# Autodesk Inventor assembly: Motor assembly V2
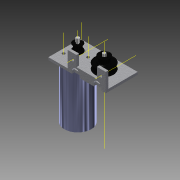
[picture p0: Inventor's stored thumbnail of the model, 180x180]
Saved by Autodesk Inventor 2013 (Build 170138000, 138)
## iProperties
Created: 2013-01-03
Part Number: Motor assembly V2
Document SubType Name: Assembly
Designer: Nico
Author: Nico
## Documents named in this file (5)
- D:\Documents\Inventor\Coil winder\IAM files\Motor assembly V2.iam
- D:\Documents\Inventor\Coil winder\IPT files\DC motor.ipt
- D:\Documents\Inventor\Coil winder\Imported Components\28-3m06m6fa6\28-3m06m6fa6.ipt
- D:\Documents\Inventor\Coil winder\Imported Components\15-3m06m6ca6\15-3m06m6ca6.ipt
- D:\Documents\Inventor\Coil winder\Imported Components\12-3m06m6ca4\12-3m06m6ca4.ipt
## Components (4 placed, 4 different names)
1. DC motor:1 — Mate:2, Mate:3, Mate:4, Mate:6, Mate:7
2. 28-3m06m6fa6:1 — Mate:2, Mate:3, Mate:5
3. 15-3m06m6ca6:1 — Mate:4, Mate:5
4. 12-3m06m6ca4:1 — Mate:6, Mate:7
## Relationships (6: Mate 6)
- Mate:2: DC motor:1 ↔ 28-3m06m6fa6:1
- Mate:3: DC motor:1 ↔ 28-3m06m6fa6:1
- Mate:4: DC motor:1 ↔ 15-3m06m6ca6:1
- Mate:5: 28-3m06m6fa6:1 ↔ 15-3m06m6ca6:1
- Mate:6: DC motor:1 ↔ 12-3m06m6ca4:1
- Mate:7: DC motor:1 ↔ 12-3m06m6ca4:1
